# Autodesk Inventor assembly: Marco_Bicicleta
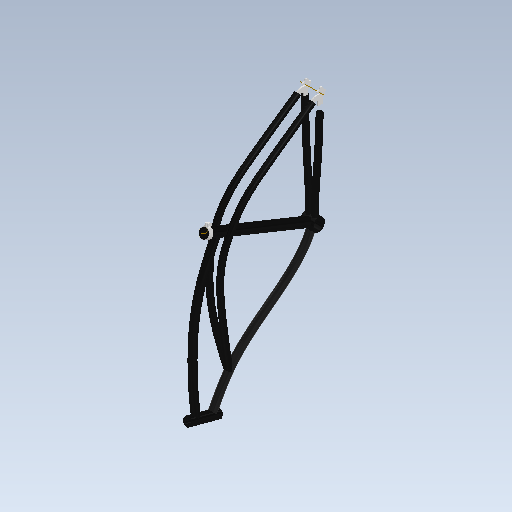
[picture p0: Inventor's stored thumbnail of the model, 512x512]
Saved by Autodesk Inventor 2021 (Build 250183000, 183)
## iProperties
Created: 2021-03-29
Part Number: Marco_Bicicleta
Document SubType Name: Assembly
Designer: j2seb
Author: j2seb
## Documents named in this file (5)
- C:\Git\Proyecto_APM\02 Inventor\Marco_Bicicleta.iam
- C:\Git\Proyecto_APM\02 Inventor\Esqueleto_estructura.ipt
- C:\Git\Proyecto_APM\02 Inventor\Marco_Bicicleta\Frame\Estructura 1617045494032.iam
- C:\Git\Proyecto_APM\02 Inventor\lamina_trasero.ipt
- C:\Git\Proyecto_APM\02 Inventor\ajuste_silin.ipt
## Components (5 placed, 4 different names)
1. Esqueleto_estructura:1 — Coincidencia:2, Coincidencia:3, Coincidencia:4, Coincidencia:5, Coincidencia:6, Coincidencia:9, Coincidencia:10
2. Estructura 1617045494032:1 [sub-assembly] — Nivelación:5
3. lamina_trasero:1 — Coincidencia:7, Coincidencia:8, Nivelación:4
4. lamina_trasero:2 — Coincidencia:12, Coincidencia:14
5. ajuste_silin:1 — Nivelación:5
## Relationships (16: Mate 13, Flush 3)
- Coincidencia:2 [Mate]: Esqueleto_estructura:1
- Coincidencia:3 [Mate]: Esqueleto_estructura:1
- Coincidencia:4 [Mate]: Esqueleto_estructura:1
- Coincidencia:5 [Mate]: Esqueleto_estructura:1
- Coincidencia:6 [Mate]: Esqueleto_estructura:1
- Nivelación:3 [Flush] (35 mm)
- Coincidencia:7 [Mate]: lamina_trasero:1
- Coincidencia:8 [Mate]: lamina_trasero:1
- Coincidencia:9 [Mate]: Esqueleto_estructura:1
- Coincidencia:10 [Mate]: Esqueleto_estructura:1
- Coincidencia:11 [Mate]
- Nivelación:4 [Flush] (36.5 mm): lamina_trasero:1
- Coincidencia:12 [Mate]: lamina_trasero:2
- Coincidencia:13 [Mate]
- Coincidencia:14 [Mate] (-36.5 mm): lamina_trasero:2
- Nivelación:5 [Flush]: Estructura 1617045494032:1 ↔ ajuste_silin:1
